# Autodesk Inventor assembly: piping
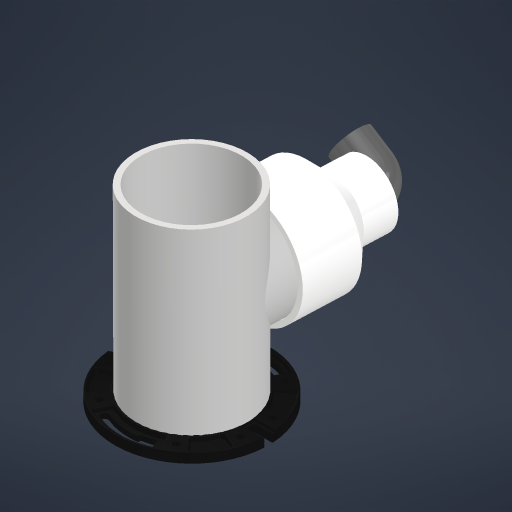
[picture p0: Inventor's stored thumbnail of the model, 512x512]
Saved by Autodesk Inventor 2024.1 (Build 281209000, 209)
## iProperties
Created: 2024-11-18
Part Number: piping
Document SubType Name: Assembly
Designer: Designer
Author: Designer
## Documents named in this file (5)
- C:\Users\Designer\Desktop\optics\Traj\piping.iam
- C:\Users\Designer\Desktop\optics\Traj\4 inch ABS Closet Flange.ipt
- C:\Users\Designer\Desktop\optics\Traj\T Junction.ipt
- C:\Users\Designer\Downloads\4 x 2 in Sch 40 Charlotte Reducer\4 x 2 in Sch 40 Charlotte Reducer.ipt
- C:\Users\Designer\Downloads\1in PVC Elbow\1in PVC Elbow.ipt
## Components (4 placed, 4 different names)
1. 4 inch ABS Closet Flange:1 — Rotational:1
2. T Junction:1 — Rotational:1, Rigid:1
3. 4 x 2 in Sch 40 Charlotte Reducer:1 — Rigid:1, Rotational:2
4. 1in PVC Elbow:1 — Rotational:2
## Relationships (3: RevoluteJoint 2, WeldJoint 1)
- Rotational:1 [RevoluteJoint]: 4 inch ABS Closet Flange:1 ↔ T Junction:1
- Rigid:1 [WeldJoint] (-50.8 mm): T Junction:1 ↔ 4 x 2 in Sch 40 Charlotte Reducer:1
- Rotational:2 [RevoluteJoint]: 4 x 2 in Sch 40 Charlotte Reducer:1 ↔ 1in PVC Elbow:1
